# Autodesk Inventor assembly: Assembly_Cube_Lens_holder_Thorlabs_AC254_v3
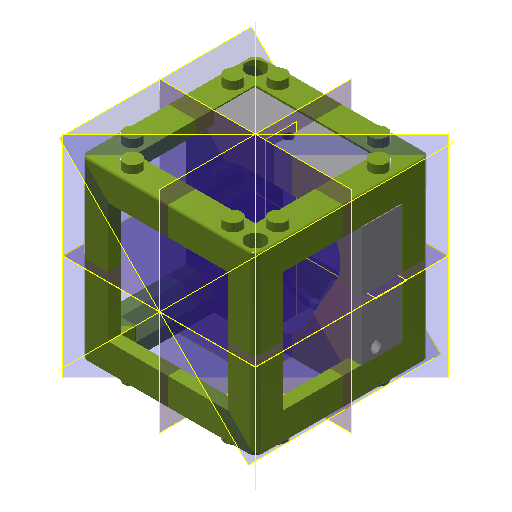
[picture p0: Inventor's stored thumbnail of the model, 512x512]
Saved by Autodesk Inventor 2022 (Build 260153000, 153)
## iProperties
Created: 2020-11-11
Part Number: Assembly_Cube_Lens_holder_Thorlabs_AC254_v3
Document SubType Name: Assembly
Designer: marsikovabarbora
Author: marsikovabarbora
## Documents named in this file (3)
- C:\Users\diederichbenedict\Dropbox\Dokumente\Promotion\PROJECTS\openUC2-CAD\INVENTOR\Assembly_Cube_Lens_holder_Thorlabs_AC254_v3.iam
- C:\Users\diederichbenedict\Dropbox\Dokumente\Promotion\PROJECTS\openUC2-CAD\INVENTOR\Assembly_Cube_empty_IM_v3.iam
- C:\Users\diederichbenedict\Dropbox\Dokumente\Promotion\PROJECTS\openUC2-CAD\INVENTOR\20_Cube_Insert_Thorlabs_SM1Tube.ipt
## Components (2 placed, 2 different names)
1. Assembly_Cube_empty_IM_v3:1 [sub-assembly] — Mate:1, Mate:2, Mate:3, Passend:12, Winkel:1
2. 20_Cube_Insert_Thorlabs_SM1Tube:1 — Passend:12, Winkel:1
## Relationships (5: Mate 4, Angle 1)
- Mate:1: Assembly_Cube_empty_IM_v3:1
- Mate:2: Assembly_Cube_empty_IM_v3:1
- Mate:3: Assembly_Cube_empty_IM_v3:1
- Passend:12 [Mate]: Assembly_Cube_empty_IM_v3:1 ↔ 20_Cube_Insert_Thorlabs_SM1Tube:1
- Winkel:1 [Angle] (180 deg): Assembly_Cube_empty_IM_v3:1 ↔ 20_Cube_Insert_Thorlabs_SM1Tube:1
